# Autodesk Inventor assembly: conjunto plato -carrete
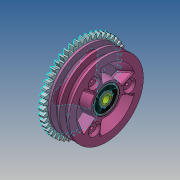
[picture p0: Inventor's stored thumbnail of the model, 180x180]
Saved by Autodesk Inventor 2017 (Build 210142000, 142)
## iProperties
Part Number: conjunto plato -carrete
Material: Genérico
Document SubType Name: Assembly
Designer: FABLAB
Author: FABLAB
## Documents named in this file (7)
- C:\Users\Leo\Documents\GitHub\actor-re-actor\models\inventor-caja\transmision Engranajes\conjunto plato-carrete.iam
- C:\Users\Leo\Documents\GitHub\actor-re-actor\models\inventor-caja\transmision Engranajes\Carrete Impreso.ipt
- C:\Users\Leo\Documents\GitHub\actor-re-actor\models\inventor-caja\transmision Engranajes\engrane acrílico C.ipt
- C:\Users\Leo\Documents\GitHub\actor-re-actor\models\inventor-caja\transmision Engranajes\conjunto plato-carrete\Design Accelerator\Conexión por perno1.iam
- C:\Users\Leo\Documents\GitHub\actor-re-actor\models\inventor-caja\Piezas\rodamiento.ipt
- C:\Users\Leo\Documents\Inventor\Content Center Files\R2017\es-ES\ANSI B18.22 M\ANSI B18.22M - 8 N.ipt
- C:\Users\Leo\Documents\GitHub\actor-re-actor\models\inventor-caja\Piezas\golilla aceilica carrete.ipt
## Components (9 placed, 6 different names)
1. Carrete Impreso:1 — Nivelación:1, Insertar:1, Insertar:2, Insertar:3
2. engrane acrílico C:1 — Nivelación:1, Nivelación:2, Coincidencia:1, Coincidencia:2, Coincidencia:3
3. rodamiento:1 — Insertar:1
4. rodamiento:2 — Insertar:2
5. Arandela plana (Métrico) 8 N:1 — Insertar:3, Insertar:4
6. golilla aceilica carrete:1 — Insertar:4
7. Conexión por perno:1 [sub-assembly] — Coincidencia:2, Coincidencia:3
8. Conexión por perno:2 [sub-assembly]
9. Conexión por perno:3 [sub-assembly]
## Component patterns: (3 elements, first: Conexión por perno:1)
## Relationships (9: Insert 4, Mate 3, Flush 2)
- Nivelación:1 [Flush]: Carrete Impreso:1 ↔ engrane acrílico C:1
- Nivelación:2 [Flush]: engrane acrílico C:1
- Coincidencia:1 [Mate]: engrane acrílico C:1
- Coincidencia:2 [Mate]: engrane acrílico C:1 ↔ Conexión por perno:1
- Coincidencia:3 [Mate]: engrane acrílico C:1 ↔ Conexión por perno:1
- Insertar:1: Carrete Impreso:1 ↔ rodamiento:1
- Insertar:2: Carrete Impreso:1 ↔ rodamiento:2
- Insertar:3: Carrete Impreso:1 ↔ Arandela plana (Métrico) 8 N:1
- Insertar:4: Arandela plana (Métrico) 8 N:1 ↔ golilla aceilica carrete:1
